# Autodesk Inventor assembly: lcall3
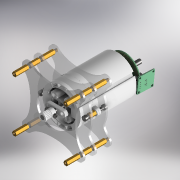
[picture p0: Inventor's stored thumbnail of the model, 180x180]
Saved by Autodesk Inventor 2018 (Build 220112000, 112)
## iProperties
Created: 2018-03-25
Part Number: lcall3
Document SubType Name: Assembly
Designer: mansu
Author: mansu
## Documents named in this file (18)
- F:\OneDrive\Documents\2018 UBC\ELEC 391\Controller\cad\release\lcall3.iam
- F:\OneDrive\Documents\2018 UBC\ELEC 391\Controller\cad\release\YawMotor.iam
- F:\OneDrive\Documents\2018 UBC\ELEC 391\Controller\cad\release\YawMotorPlate.ipt
- F:\OneDrive\Documents\2018 UBC\ELEC 391\Controller\cad\release\Fasteners\StandoffM4x20B.ipt
- F:\OneDrive\Documents\2018 UBC\ELEC 391\Controller\cad\release\Fasteners\StandoffM4x10A.ipt
- F:\OneDrive\Documents\2018 UBC\ELEC 391\Controller\cad\release\Fasteners\StandoffM4x15B.ipt
- F:\OneDrive\Documents\2018 UBC\ELEC 391\Controller\cad\release\EncoderWheelYaw.ipt
- F:\OneDrive\Documents\2018 UBC\ELEC 391\Controller\cad\release\EncoderWheelAdapter.ipt
- C:\Users\mansu\Documents\Inventor\Content Center Files\R2018\en-US\AS 1420\AS 1420 - 1973 - M3 x 8.ipt
- C:\Users\mansu\Documents\Inventor\Content Center Files\R2018\en-US\AS 1474(1)\AS 1474 - M3(1).ipt
- C:\Users\mansu\Documents\Inventor\Content Center Files\R2018\en-US\AS 1420\AS 1420 - 1973 - M3 x 12.ipt
- F:\OneDrive\Documents\2018 UBC\ELEC 391\Controller\cad\release\GT2Yaw.ipt
- C:\Users\mansu\Documents\Inventor\Content Center Files\R2018\en-US\AS 1420\AS 1420 - 1973 - M3 x 14.ipt
- C:\Users\mansu\Documents\Inventor\Content Center Files\R2018\en-US\AS 1420\AS 1420 - 1973 - M4 x 16.ipt
- C:\Users\mansu\Documents\Inventor\Content Center Files\R2018\en-US\AS 1420\AS 1420 - 1973 - M4 x 8.ipt
- F:\OneDrive\Documents\2018 UBC\ELEC 391\Controller\cad\release\EncoderPCBAssembly.iam
- F:\OneDrive\Documents\2018 UBC\ELEC 391\Controller\cad\release\YawBottomPlate.ipt
- F:\OneDrive\Documents\2018 UBC\ELEC 391\Controller\cad\release\Magnet6010.ipt
## Components (40 placed, 17 different names)
1. YawMotor:1 [sub-assembly] — Mate:7, Mate:8, Mate:11, Mate:12, Mate:13, Mate:14, Mate:21, Mate:24, Flush:1, Mate:30, Mate:31, Flush:2, Mate:32, Mate:33, Flush:3, Mate:34, Mate:35, Flush:4, Mate:36, Mate:37, Flush:5, Mate:38, Mate:39, Flush:6, Mate:40, Mate:41, Flush:7
2. YawMotorPlate:1 — Mate:5, Mate:8, Mate:10, Mate:27, Mate:28, Insert:15
3. YawMotorPlate:2 — Mate:6, Mate:7, Insert:3, Insert:4, Mate:11, Insert:5, Insert:6, Insert:7, Insert:8, Insert:9, Insert:10, Insert:11, Insert:12, Insert:16, Insert:17
4. EncoderWheelYaw:1 — Mate:13, Mate:15, Mate:16, Insert:13, Insert:14, Mate:21
5. EncoderWheelAdapter:1 — Mate:14, Mate:15, Mate:16, Mate:18, Mate:20, Mate:22, Tangent:1, Tangent:2
6. GT2Yaw:1 — Mate:24, Flush:1, Mate:25, Tangent:3, Tangent:4
7. AS 1420 - Metric M3 x 14:1 — Mate:25, Tangent:3, Mate:26
8. AS 1474 - Metric M3:4 — Mate:26, Tangent:4
9. AS 1420 - Metric M4 x 16:1 — Mate:27, Mate:28
10. AS 1420 - Metric M4 x 16:2 — Insert:15
11. AS 1420 - Metric M4 x 8:1 — Insert:16
12. AS 1420 - Metric M4 x 8:2 — Insert:17
13. EncoderPCBAssembly:1 [sub-assembly]
14. YawBottomPlate:1 — Insert:18, Mate:29, Insert:19, Insert:20, Insert:21, Insert:22
15. StandoffM4x20B:11 — Insert:20
16. StandoffM4x20B:12 — Insert:21
17. StandoffM4x20B:13 — Insert:22
18. StandoffM4x20B:14 — Insert:19
19. Magnet6010:1 — Mate:34, Mate:35, Flush:4
20. Magnet6010:2 — Mate:32, Mate:33, Flush:3
21. Magnet6010:3 — Mate:30, Mate:31, Flush:2
22. Magnet6010:4 — Mate:38, Mate:39, Flush:6
23. Magnet6010:5 — Mate:36, Mate:37, Flush:5
24. Magnet6010:6 — Mate:40, Mate:41, Flush:7
25. StandoffM4x20B:1 — Insert:4, Mate:10
26. StandoffM4x15B:2 — Insert:3
27. StandoffM4x10A:1 — Insert:5, Mate:12
28. StandoffM4x10A:2 — Insert:6
29. StandoffM4x15B:4 — Insert:7, Mate:29
30. StandoffM4x20B:6 — Insert:8
31. StandoffM4x20B:7 — Insert:12
32. StandoffM4x15B:1 — Insert:11, Insert:18
33. StandoffM4x15B:3 — Insert:9
34. StandoffM4x20B:10 — Insert:10
35. AS 1420 - Metric M3 x 8:1 — Insert:13, Mate:17
36. AS 1420 - Metric M3 x 8:2 — Insert:14, Mate:19
37. AS 1474 - Metric M3:1 — Mate:17, Mate:18
38. AS 1474 - Metric M3:2 — Mate:19, Mate:20
39. AS 1420 - Metric M3 x 12:1 — Mate:22, Tangent:1, Mate:23
40. AS 1474 - Metric M3:3 — Mate:23, Tangent:2
## Relationships (67: Mate 36, Insert 20, Flush 7, Tangent 4)
- Mate:5: YawMotorPlate:1
- Mate:6: YawMotorPlate:2
- Mate:7: YawMotor:1 ↔ YawMotorPlate:2
- Mate:8: YawMotor:1 ↔ YawMotorPlate:1
- Insert:3: YawMotorPlate:2 ↔ StandoffM4x15B:2
- Insert:4: YawMotorPlate:2 ↔ StandoffM4x20B:1
- Mate:10 (0.1 mm): YawMotorPlate:1 ↔ StandoffM4x20B:1
- Mate:11: YawMotor:1 ↔ YawMotorPlate:2
- Insert:5: YawMotorPlate:2 ↔ StandoffM4x10A:1
- Mate:12: YawMotor:1 ↔ StandoffM4x10A:1
- Insert:6: YawMotorPlate:2 ↔ StandoffM4x10A:2
- Insert:7: YawMotorPlate:2 ↔ StandoffM4x15B:4
- Insert:8: YawMotorPlate:2 ↔ StandoffM4x20B:6
- Insert:9: YawMotorPlate:2 ↔ StandoffM4x15B:3
- Insert:10: YawMotorPlate:2 ↔ StandoffM4x20B:10
- Insert:11: YawMotorPlate:2 ↔ StandoffM4x15B:1
- Insert:12: YawMotorPlate:2 ↔ StandoffM4x20B:7
- Mate:13: YawMotor:1 ↔ EncoderWheelYaw:1
- Mate:14: YawMotor:1 ↔ EncoderWheelAdapter:1
- Mate:15: EncoderWheelYaw:1 ↔ EncoderWheelAdapter:1
- Mate:16 (0.1 mm): EncoderWheelYaw:1 ↔ EncoderWheelAdapter:1
- Insert:13: EncoderWheelYaw:1 ↔ AS 1420 - Metric M3 x 8:1
- Insert:14: EncoderWheelYaw:1 ↔ AS 1420 - Metric M3 x 8:2
- Mate:17: AS 1420 - Metric M3 x 8:1 ↔ AS 1474 - Metric M3:1
- Mate:18: EncoderWheelAdapter:1 ↔ AS 1474 - Metric M3:1
- Mate:19: AS 1420 - Metric M3 x 8:2 ↔ AS 1474 - Metric M3:2
- Mate:20: EncoderWheelAdapter:1 ↔ AS 1474 - Metric M3:2
- Mate:21 (10 mm): YawMotor:1 ↔ EncoderWheelYaw:1
- Mate:22: EncoderWheelAdapter:1 ↔ AS 1420 - Metric M3 x 12:1
- Tangent:1 (0.1 mm): EncoderWheelAdapter:1 ↔ AS 1420 - Metric M3 x 12:1
- Mate:23: AS 1420 - Metric M3 x 12:1 ↔ AS 1474 - Metric M3:3
- Tangent:2 (0.1 mm): EncoderWheelAdapter:1 ↔ AS 1474 - Metric M3:3
- Mate:24: YawMotor:1 ↔ GT2Yaw:1
- Flush:1: YawMotor:1 ↔ GT2Yaw:1
- Mate:25: GT2Yaw:1 ↔ AS 1420 - Metric M3 x 14:1
- Tangent:3 (0.1 mm): GT2Yaw:1 ↔ AS 1420 - Metric M3 x 14:1
- Mate:26: AS 1420 - Metric M3 x 14:1 ↔ AS 1474 - Metric M3:4
- Tangent:4 (0.1 mm): GT2Yaw:1 ↔ AS 1474 - Metric M3:4
- Mate:27: YawMotorPlate:1 ↔ AS 1420 - Metric M4 x 16:1
- Mate:28: YawMotorPlate:1 ↔ AS 1420 - Metric M4 x 16:1
- Insert:15: YawMotorPlate:1 ↔ AS 1420 - Metric M4 x 16:2
- Insert:16: YawMotorPlate:2 ↔ AS 1420 - Metric M4 x 8:1
- Insert:17: YawMotorPlate:2 ↔ AS 1420 - Metric M4 x 8:2
- Insert:18 (0.1 mm): YawBottomPlate:1 ↔ StandoffM4x15B:1
- Mate:29: YawBottomPlate:1 ↔ StandoffM4x15B:4
- Insert:19: YawBottomPlate:1 ↔ StandoffM4x20B:14
- Insert:20: YawBottomPlate:1 ↔ StandoffM4x20B:11
- Insert:21: YawBottomPlate:1 ↔ StandoffM4x20B:12
- Insert:22: YawBottomPlate:1 ↔ StandoffM4x20B:13
- Mate:30: YawMotor:1 ↔ Magnet6010:3
- Mate:31: YawMotor:1 ↔ Magnet6010:3
- Flush:2 (5 mm): YawMotor:1 ↔ Magnet6010:3
- Mate:32: YawMotor:1 ↔ Magnet6010:2
- Mate:33: YawMotor:1 ↔ Magnet6010:2
- Flush:3 (5 mm): YawMotor:1 ↔ Magnet6010:2
- Mate:34: YawMotor:1 ↔ Magnet6010:1
- Mate:35: YawMotor:1 ↔ Magnet6010:1
- Flush:4 (5 mm): YawMotor:1 ↔ Magnet6010:1
- Mate:36: YawMotor:1 ↔ Magnet6010:5
- Mate:37: YawMotor:1 ↔ Magnet6010:5
- Flush:5 (5 mm): YawMotor:1 ↔ Magnet6010:5
- Mate:38: YawMotor:1 ↔ Magnet6010:4
- Mate:39: YawMotor:1 ↔ Magnet6010:4
- Flush:6 (5 mm): YawMotor:1 ↔ Magnet6010:4
- Mate:40: YawMotor:1 ↔ Magnet6010:6
- Mate:41: YawMotor:1 ↔ Magnet6010:6
- Flush:7 (5 mm): YawMotor:1 ↔ Magnet6010:6
